# Autodesk Inventor assembly: frame_1_0
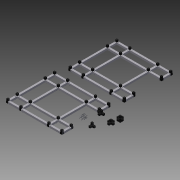
[picture p0: Inventor's stored thumbnail of the model, 180x180]
Saved by Autodesk Inventor 2011 (Build 150239000, 239)
## iProperties
Created: 2013-01-19
Part Number: frame_1_0
Document SubType Name: Assembly
Designer: Christopher
Author: Christopher
## Documents named in this file (30)
- F:\Users\Christopher\Documents\GitHub\2013CAD\2013 robot\forklift\robot_frame\frame_1_0.iam
- F:\Users\Christopher\Documents\GitHub\2013CAD\2013 robot\forklift\robot_frame\tubes_layer1\tube_m_f_in_cross.ipt
- F:\Users\Christopher\Documents\GitHub\2013CAD\2013 robot\forklift\Misc parts\3-way corner.ipt
- F:\Users\Christopher\Documents\GitHub\2013CAD\2013 robot\forklift\Misc parts\4-way corner.ipt
- F:\Users\Christopher\Documents\GitHub\2013CAD\2013 robot\forklift\Misc parts\5-way corner.ipt
- F:\Users\Christopher\Documents\GitHub\2013CAD\2013 robot\forklift\Misc parts\6-way corner.ipt
- F:\Users\Christopher\Documents\GitHub\2013CAD\2013 robot\forklift\Misc parts\1.5_bolt_.25_20.ipt
- F:\Users\Christopher\Documents\GitHub\2013CAD\2013 robot\forklift\robot_frame\tubes_layer1\tube_m_b_in_cross.ipt
- F:\Users\Christopher\Documents\GitHub\2013CAD\2013 robot\forklift\robot_frame\tubes_layer1\tube_m_r_in_mid.ipt
- F:\Users\Christopher\Documents\GitHub\2013CAD\2013 robot\forklift\robot_frame\tubes_layer1\tube_r_b_in.ipt
- F:\Users\Christopher\Documents\GitHub\2013CAD\2013 robot\forklift\robot_frame\tubes_layer1\tube_r_f_in.ipt
- F:\Users\Christopher\Documents\GitHub\2013CAD\2013 robot\forklift\robot_frame\tubes_layer1\tube_m_r_out_center.ipt
- F:\Users\Christopher\Documents\GitHub\2013CAD\2013 robot\forklift\robot_frame\tubes_layer1\tube_b_r_in_wheel.ipt
- F:\Users\Christopher\Documents\GitHub\2013CAD\2013 robot\forklift\robot_frame\tubes_layer1\tube_r_b_out.ipt
- F:\Users\Christopher\Documents\GitHub\2013CAD\2013 robot\forklift\robot_frame\tubes_layer1\tube_b_r_wheel.ipt
- F:\Users\Christopher\Documents\GitHub\2013CAD\2013 robot\forklift\robot_frame\tubes_layer1\tube_f_r_in_wheel.ipt
- F:\Users\Christopher\Documents\GitHub\2013CAD\2013 robot\forklift\robot_frame\tubes_layer1\tube_f_r_out_wheel.ipt
- F:\Users\Christopher\Documents\GitHub\2013CAD\2013 robot\forklift\robot_frame\tubes_layer1\tube_r_f_out.ipt
- F:\Users\Christopher\Documents\GitHub\2013CAD\2013 robot\forklift\robot_frame\tubes_layer1\tube_m_b_out_back.ipt
- F:\Users\Christopher\Documents\GitHub\2013CAD\2013 robot\forklift\robot_frame\tubes_layer1\tube_b_l_in_wheel.ipt
- F:\Users\Christopher\Documents\GitHub\2013CAD\2013 robot\forklift\robot_frame\tubes_layer1\tube_m_l_in.ipt
- F:\Users\Christopher\Documents\GitHub\2013CAD\2013 robot\forklift\robot_frame\tubes_layer1\tube_f_l_in_wheel.ipt
- F:\Users\Christopher\Documents\GitHub\2013CAD\2013 robot\forklift\robot_frame\tubes_layer1\tube_l_f_out.ipt
- F:\Users\Christopher\Documents\GitHub\2013CAD\2013 robot\forklift\robot_frame\tubes_layer1\tube_l_f_in.ipt
- F:\Users\Christopher\Documents\GitHub\2013CAD\2013 robot\forklift\robot_frame\tubes_layer1\tube_l_b_in.ipt
- F:\Users\Christopher\Documents\GitHub\2013CAD\2013 robot\forklift\robot_frame\tubes_layer1\tube_l_b_out.ipt
- F:\Users\Christopher\Documents\GitHub\2013CAD\2013 robot\forklift\robot_frame\tubes_layer1\tube_b_l_out_wheel.ipt
- F:\Users\Christopher\Documents\GitHub\2013CAD\2013 robot\forklift\robot_frame\tubes_layer1\tube_f_l_out_wheel.ipt
- F:\Users\Christopher\Documents\GitHub\2013CAD\2013 robot\forklift\robot_frame\tubes_layer1\tube_m_l_out.ipt
- F:\Users\Christopher\Documents\GitHub\2013CAD\2013 robot\forklift\robot_frame\tubes_layer2\frame_level1_temp.iam
## Components (106 placed, 29 different names)
1. tube_m_f_in_cross:1 — Insert:1, Insert:2, Mate:2, Insert:3, Insert:4, Mate:3
2. 3-way corner:1
3. 4-way corner:1
4. 5-way corner:1
5. 6-way corner:1
6. 5-way corner:2 — Insert:1, Mate:3, Mate:4, Insert:5, Mate:8, Insert:13, Mate:18, Insert:35
7. 1.5_bolt_.25_20:1 — Insert:4
8. 5-way corner:3 — Mate:5, Insert:7, Mate:6, Insert:9, Mate:7, Insert:11, Mate:12, Insert:23
9. 1.5_bolt_.25_20:2 — Insert:2
10. 5-way corner:4 — Mate:2, Insert:3, Mate:30, Insert:58, Mate:31, Insert:62, Mate:34, Insert:70
11. 1.5_bolt_.25_20:3 — Insert:12
12. tube_m_b_in_cross:1 — Mate:6, Insert:9, Insert:10, Mate:25, Insert:49, Insert:51
13. tube_m_r_in_mid:1 — Mate:4, Insert:5, Insert:6, Mate:5, Insert:7, Insert:8
14. 1.5_bolt_.25_20:4 — Insert:6
15. 1.5_bolt_.25_20:5 — Insert:22
16. 1.5_bolt_.25_20:6 — Insert:26
17. 1.5_bolt_.25_20:7 — Insert:28
18. 1.5_bolt_.25_20:8 — Insert:30
19. 1.5_bolt_.25_20:10 — Insert:8
20. 1.5_bolt_.25_20:11 — Insert:10
21. 1.5_bolt_.25_20:12 — Insert:14
22. 1.5_bolt_.25_20:13 — Insert:16
23. 1.5_bolt_.25_20:14 — Insert:18
24. 1.5_bolt_.25_20:15 — Insert:19
25. 1.5_bolt_.25_20:16 — Insert:24
26. tube_r_b_in:1 — Mate:7, Insert:11, Insert:12, Mate:11, Insert:19, Insert:20
27. tube_r_f_in:1 — Mate:8, Insert:13, Insert:14, Mate:9, Insert:15, Insert:16
28. tube_m_r_out_center:1 — Mate:10, Insert:17, Insert:18, Insert:21, Flush:1, Insert:22
29. 4-way corner:2 — Mate:9, Insert:15, Mate:10, Insert:17, Mate:20, Insert:39
30. 4-way corner:3 — Mate:11, Insert:20, Insert:21, Flush:1, Mate:17, Insert:32
31. 3-way corner:2 — Mate:15, Insert:29, Mate:16, Insert:31
32. 4-way corner:4 — Mate:13, Insert:25, Mate:14, Insert:27, Mate:24, Insert:47
33. tube_b_r_in_wheel:1 — Mate:12, Insert:23, Insert:24, Mate:13, Insert:25, Insert:26
34. tube_r_b_out:1 — Mate:14, Insert:27, Insert:28, Mate:15, Insert:29, Insert:30
35. 1.5_bolt_.25_20:17 — Insert:48
36. 1.5_bolt_.25_20:18 — Insert:56
37. 1.5_bolt_.25_20:19 — Insert:42
38. 1.5_bolt_.25_20:20 — Insert:40
39. 1.5_bolt_.25_20:21 — Insert:36
40. 1.5_bolt_.25_20:22 — Insert:51
41. 1.5_bolt_.25_20:23 — Insert:52
42. 1.5_bolt_.25_20:24 — Insert:33
43. 1.5_bolt_.25_20:25 — Insert:45
44. 1.5_bolt_.25_20:26 — Insert:38
45. 1.5_bolt_.25_20:27 — Insert:46
46. 1.5_bolt_.25_20:28 — Insert:34
47. tube_b_r_wheel:1 — Mate:16, Mate:17, Insert:31, Insert:32, Insert:33, Insert:34
48. tube_f_r_in_wheel:1 — Mate:18, Insert:35, Insert:36, Mate:19, Insert:37, Insert:38
49. tube_f_r_out_wheel:1 — Mate:20, Insert:39, Insert:40, Mate:21, Insert:41, Insert:42
50. 3-way corner:3 — Mate:21, Insert:41, Mate:23, Insert:43
51. 3-way corner:4 — Mate:19, Insert:37, Mate:22, Insert:44
52. tube_r_f_out:1 — Mate:22, Mate:23, Insert:43, Insert:44, Insert:45, Insert:46
53. tube_m_b_out_back:1 — Mate:24, Insert:47, Insert:48, Insert:52, Mate:26, Insert:53
54. 5-way corner:5 — Mate:25, Insert:49, Mate:27, Insert:55, Mate:29, Insert:59, Mate:35, Insert:71
55. 4-way corner:5 — Mate:26, Insert:53, Mate:28, Insert:54, Mate:36, Insert:72
56. tube_b_l_in_wheel:1 — Mate:27, Mate:28, Insert:54, Insert:55, Insert:56, Insert:57
57. 1.5_bolt_.25_20:29
58. 1.5_bolt_.25_20:30 — Insert:67
59. 1.5_bolt_.25_20:31 — Insert:69
60. 1.5_bolt_.25_20:32 — Insert:79
61. 1.5_bolt_.25_20:33 — Insert:78
62. 1.5_bolt_.25_20:34 — Insert:63
63. 1.5_bolt_.25_20:35 — Insert:57
64. 1.5_bolt_.25_20:36 — Insert:66
65. 1.5_bolt_.25_20:37 — Insert:61
66. 1.5_bolt_.25_20:38 — Insert:60
67. tube_m_l_in:1 — Mate:29, Mate:30, Insert:58, Insert:59, Insert:60, Insert:61
68. tube_f_l_in_wheel:1 — Mate:31, Insert:62, Insert:63, Mate:32, Insert:64, Insert:67
69. 3-way corner:5 — Mate:32, Insert:64, Flush:2, Insert:65
70. tube_l_f_out:1 — Flush:2, Insert:65, Insert:66, Mate:33, Insert:68, Insert:69
71. 3-way corner:6 — Mate:33, Insert:68, Mate:42, Insert:83
72. tube_l_f_in:1 — Mate:34, Insert:70, Flush:3, Insert:73, Insert:76, Insert:77
73. tube_l_b_in:1 — Mate:35, Insert:71, Flush:4, Insert:74, Insert:78, Insert:93
74. tube_l_b_out:1 — Mate:36, Insert:72, Flush:5, Insert:75, Insert:79, Insert:80
75. 4-way corner:6 — Flush:3, Insert:73, Mate:40, Mate:41, Insert:84, Insert:85
76. 4-way corner:7 — Flush:4, Insert:74, Mate:38, Insert:81, Mate:39, Insert:86, Insert:87
77. 3-way corner:7 — Flush:5, Insert:75, Mate:37, Insert:82, Insert:88
78. 1.5_bolt_.25_20:39 — Insert:76
79. 1.5_bolt_.25_20:40 — Insert:80
80. 1.5_bolt_.25_20:41 — Insert:77
81. 1.5_bolt_.25_20:42 — Insert:93
82. 1.5_bolt_.25_20:43 — Insert:91
83. 1.5_bolt_.25_20:44 — Insert:92
84. 1.5_bolt_.25_20:45 — Insert:90
85. 1.5_bolt_.25_20:46 — Insert:89
86. tube_b_l_out_wheel:1 — Mate:37, Mate:38, Insert:81, Insert:82, Insert:87, Insert:88, Insert:94, Insert:95
87. tube_f_l_out_wheel:1 — Mate:41, Mate:42, Insert:83, Insert:84, Insert:89, Insert:90
88. tube_m_l_out:1 — Mate:39, Mate:40, Insert:85, Insert:86, Insert:91, Insert:92
89. 1.5_bolt_.25_20:47
90. 1.5_bolt_.25_20:48
91. 1.5_bolt_.25_20:49
92. 1.5_bolt_.25_20:50 — Insert:94
93. 1.5_bolt_.25_20:51 — Insert:95
94. 1.5_bolt_.25_20:52
95. 1.5_bolt_.25_20:53
96. 1.5_bolt_.25_20:54
97. 1.5_bolt_.25_20:55
98. 1.5_bolt_.25_20:56
99. 1.5_bolt_.25_20:57
100. 1.5_bolt_.25_20:58
101. 1.5_bolt_.25_20:59
102. 1.5_bolt_.25_20:60
103. 1.5_bolt_.25_20:61
104. 1.5_bolt_.25_20:62
105. 1.5_bolt_.25_20:63
106. frame_level1_temp:1 [sub-assembly]
## Relationships (140: Insert 94, Mate 41, Flush 5)
- Insert:1: tube_m_f_in_cross:1 ↔ 5-way corner:2
- Insert:2: tube_m_f_in_cross:1 ↔ 1.5_bolt_.25_20:2
- Mate:2: tube_m_f_in_cross:1 ↔ 5-way corner:4
- Insert:3: tube_m_f_in_cross:1 ↔ 5-way corner:4
- Insert:4: tube_m_f_in_cross:1 ↔ 1.5_bolt_.25_20:1
- Mate:3: tube_m_f_in_cross:1 ↔ 5-way corner:2
- Mate:4: 5-way corner:2 ↔ tube_m_r_in_mid:1
- Insert:5: 5-way corner:2 ↔ tube_m_r_in_mid:1
- Insert:6: tube_m_r_in_mid:1 ↔ 1.5_bolt_.25_20:4
- Mate:5: 5-way corner:3 ↔ tube_m_r_in_mid:1
- Insert:7: 5-way corner:3 ↔ tube_m_r_in_mid:1
- Insert:8: tube_m_r_in_mid:1 ↔ 1.5_bolt_.25_20:10
- Mate:6: 5-way corner:3 ↔ tube_m_b_in_cross:1
- Insert:9: 5-way corner:3 ↔ tube_m_b_in_cross:1
- Insert:10: tube_m_b_in_cross:1 ↔ 1.5_bolt_.25_20:11
- Mate:7: 5-way corner:3 ↔ tube_r_b_in:1
- Insert:11: 5-way corner:3 ↔ tube_r_b_in:1
- Insert:12: 1.5_bolt_.25_20:3 ↔ tube_r_b_in:1
- Mate:8: 5-way corner:2 ↔ tube_r_f_in:1
- Insert:13: 5-way corner:2 ↔ tube_r_f_in:1
- Insert:14: 1.5_bolt_.25_20:12 ↔ tube_r_f_in:1
- Mate:9: tube_r_f_in:1 ↔ 4-way corner:2
- Insert:15: tube_r_f_in:1 ↔ 4-way corner:2
- Mate:10: tube_m_r_out_center:1 ↔ 4-way corner:2
- Insert:16: 1.5_bolt_.25_20:13 ↔ tube_r_f_in:1
- Insert:17: tube_m_r_out_center:1 ↔ 4-way corner:2
- Insert:18: 1.5_bolt_.25_20:14 ↔ tube_m_r_out_center:1
- Mate:11: tube_r_b_in:1 ↔ 4-way corner:3
- Insert:19: 1.5_bolt_.25_20:15 ↔ tube_r_b_in:1
- Insert:20: tube_r_b_in:1 ↔ 4-way corner:3
- Insert:21: tube_m_r_out_center:1 ↔ 4-way corner:3
- Flush:1: tube_m_r_out_center:1 ↔ 4-way corner:3
- Insert:22: 1.5_bolt_.25_20:5 ↔ tube_m_r_out_center:1
- Mate:12: 5-way corner:3 ↔ tube_b_r_in_wheel:1
- Insert:23: 5-way corner:3 ↔ tube_b_r_in_wheel:1
- Insert:24: 1.5_bolt_.25_20:16 ↔ tube_b_r_in_wheel:1
- Mate:13: 4-way corner:4 ↔ tube_b_r_in_wheel:1
- Insert:25: 4-way corner:4 ↔ tube_b_r_in_wheel:1
- Insert:26: 1.5_bolt_.25_20:6 ↔ tube_b_r_in_wheel:1
- Mate:14: 4-way corner:4 ↔ tube_r_b_out:1
- Insert:27: 4-way corner:4 ↔ tube_r_b_out:1
- Insert:28: 1.5_bolt_.25_20:7 ↔ tube_r_b_out:1
- Mate:15: 3-way corner:2 ↔ tube_r_b_out:1
- Insert:29: 3-way corner:2 ↔ tube_r_b_out:1
- Insert:30: 1.5_bolt_.25_20:8 ↔ tube_r_b_out:1
- Mate:16: 3-way corner:2 ↔ tube_b_r_wheel:1
- Mate:17: 4-way corner:3 ↔ tube_b_r_wheel:1
- Insert:31: 3-way corner:2 ↔ tube_b_r_wheel:1
- Insert:32: 4-way corner:3 ↔ tube_b_r_wheel:1
- Insert:33: 1.5_bolt_.25_20:24 ↔ tube_b_r_wheel:1
- Insert:34: 1.5_bolt_.25_20:28 ↔ tube_b_r_wheel:1
- Mate:18: 5-way corner:2 ↔ tube_f_r_in_wheel:1
- Insert:35: 5-way corner:2 ↔ tube_f_r_in_wheel:1
- Insert:36: 1.5_bolt_.25_20:21 ↔ tube_f_r_in_wheel:1
- Mate:19: tube_f_r_in_wheel:1 ↔ 3-way corner:4
- Insert:37: tube_f_r_in_wheel:1 ↔ 3-way corner:4
- Insert:38: 1.5_bolt_.25_20:26 ↔ tube_f_r_in_wheel:1
- Mate:20: 4-way corner:2 ↔ tube_f_r_out_wheel:1
- Insert:39: 4-way corner:2 ↔ tube_f_r_out_wheel:1
- Insert:40: 1.5_bolt_.25_20:20 ↔ tube_f_r_out_wheel:1
- Mate:21: tube_f_r_out_wheel:1 ↔ 3-way corner:3
- Insert:41: tube_f_r_out_wheel:1 ↔ 3-way corner:3
- Insert:42: 1.5_bolt_.25_20:19 ↔ tube_f_r_out_wheel:1
- Mate:22: 3-way corner:4 ↔ tube_r_f_out:1
- Mate:23: 3-way corner:3 ↔ tube_r_f_out:1
- Insert:43: 3-way corner:3 ↔ tube_r_f_out:1
- Insert:44: 3-way corner:4 ↔ tube_r_f_out:1
- Insert:45: 1.5_bolt_.25_20:25 ↔ tube_r_f_out:1
- Insert:46: 1.5_bolt_.25_20:27 ↔ tube_r_f_out:1
- Mate:24: 4-way corner:4 ↔ tube_m_b_out_back:1
- Insert:47: 4-way corner:4 ↔ tube_m_b_out_back:1
- Insert:48: 1.5_bolt_.25_20:17 ↔ tube_m_b_out_back:1
- Mate:25: tube_m_b_in_cross:1 ↔ 5-way corner:5
- Insert:49: tube_m_b_in_cross:1 ↔ 5-way corner:5
- Insert:51: tube_m_b_in_cross:1 ↔ 1.5_bolt_.25_20:22
- Insert:52: 1.5_bolt_.25_20:23 ↔ tube_m_b_out_back:1
- Mate:26: tube_m_b_out_back:1 ↔ 4-way corner:5
- Insert:53: tube_m_b_out_back:1 ↔ 4-way corner:5
- Mate:27: 5-way corner:5 ↔ tube_b_l_in_wheel:1
- Mate:28: 4-way corner:5 ↔ tube_b_l_in_wheel:1
- Insert:54: 4-way corner:5 ↔ tube_b_l_in_wheel:1
- Insert:55: 5-way corner:5 ↔ tube_b_l_in_wheel:1
- Insert:56: 1.5_bolt_.25_20:18 ↔ tube_b_l_in_wheel:1
- Insert:57: tube_b_l_in_wheel:1 ↔ 1.5_bolt_.25_20:35
- Mate:29: 5-way corner:5 ↔ tube_m_l_in:1
- Mate:30: 5-way corner:4 ↔ tube_m_l_in:1
- Insert:58: 5-way corner:4 ↔ tube_m_l_in:1
- Insert:59: 5-way corner:5 ↔ tube_m_l_in:1
- Insert:60: 1.5_bolt_.25_20:38 ↔ tube_m_l_in:1
- Insert:61: 1.5_bolt_.25_20:37 ↔ tube_m_l_in:1
- Mate:31: 5-way corner:4 ↔ tube_f_l_in_wheel:1
- Insert:62: 5-way corner:4 ↔ tube_f_l_in_wheel:1
- Insert:63: 1.5_bolt_.25_20:34 ↔ tube_f_l_in_wheel:1
- Mate:32: tube_f_l_in_wheel:1 ↔ 3-way corner:5
- Insert:64: tube_f_l_in_wheel:1 ↔ 3-way corner:5
- Flush:2: 3-way corner:5 ↔ tube_l_f_out:1
- Insert:65: 3-way corner:5 ↔ tube_l_f_out:1
- Insert:66: 1.5_bolt_.25_20:36 ↔ tube_l_f_out:1
- Insert:67: 1.5_bolt_.25_20:30 ↔ tube_f_l_in_wheel:1
- Mate:33: tube_l_f_out:1 ↔ 3-way corner:6
- Insert:68: tube_l_f_out:1 ↔ 3-way corner:6
- Insert:69: 1.5_bolt_.25_20:31 ↔ tube_l_f_out:1
- Mate:34: 5-way corner:4 ↔ tube_l_f_in:1
- Mate:35: 5-way corner:5 ↔ tube_l_b_in:1
- Mate:36: 4-way corner:5 ↔ tube_l_b_out:1
- Insert:70: 5-way corner:4 ↔ tube_l_f_in:1
- Insert:71: 5-way corner:5 ↔ tube_l_b_in:1
- Insert:72: 4-way corner:5 ↔ tube_l_b_out:1
- Flush:3: tube_l_f_in:1 ↔ 4-way corner:6
- Flush:4: tube_l_b_in:1 ↔ 4-way corner:7
- Flush:5: tube_l_b_out:1 ↔ 3-way corner:7
- Insert:73: tube_l_f_in:1 ↔ 4-way corner:6
- Insert:74: tube_l_b_in:1 ↔ 4-way corner:7
- Insert:75: tube_l_b_out:1 ↔ 3-way corner:7
- Insert:76: tube_l_f_in:1 ↔ 1.5_bolt_.25_20:39
- Insert:77: tube_l_f_in:1 ↔ 1.5_bolt_.25_20:41
- Insert:78: 1.5_bolt_.25_20:33 ↔ tube_l_b_in:1
- Insert:79: 1.5_bolt_.25_20:32 ↔ tube_l_b_out:1
- Insert:80: tube_l_b_out:1 ↔ 1.5_bolt_.25_20:40
- Mate:37: 3-way corner:7 ↔ tube_b_l_out_wheel:1
- Mate:38: 4-way corner:7 ↔ tube_b_l_out_wheel:1
- Insert:81: 4-way corner:7 ↔ tube_b_l_out_wheel:1
- Insert:82: 3-way corner:7 ↔ tube_b_l_out_wheel:1
- Mate:39: 4-way corner:7 ↔ tube_m_l_out:1
- Mate:40: 4-way corner:6 ↔ tube_m_l_out:1
- Mate:41: 4-way corner:6 ↔ tube_f_l_out_wheel:1
- Mate:42: 3-way corner:6 ↔ tube_f_l_out_wheel:1
- Insert:83: 3-way corner:6 ↔ tube_f_l_out_wheel:1
- Insert:84: 4-way corner:6 ↔ tube_f_l_out_wheel:1
- Insert:85: 4-way corner:6 ↔ tube_m_l_out:1
- Insert:86: 4-way corner:7 ↔ tube_m_l_out:1
- Insert:87: 4-way corner:7 ↔ tube_b_l_out_wheel:1
- Insert:88: 3-way corner:7 ↔ tube_b_l_out_wheel:1
- Insert:89: 1.5_bolt_.25_20:46 ↔ tube_f_l_out_wheel:1
- Insert:90: 1.5_bolt_.25_20:45 ↔ tube_f_l_out_wheel:1
- Insert:91: 1.5_bolt_.25_20:43 ↔ tube_m_l_out:1
- Insert:92: 1.5_bolt_.25_20:44 ↔ tube_m_l_out:1
- Insert:93: tube_l_b_in:1 ↔ 1.5_bolt_.25_20:42
- Insert:94: tube_b_l_out_wheel:1 ↔ 1.5_bolt_.25_20:50
- Insert:95: tube_b_l_out_wheel:1 ↔ 1.5_bolt_.25_20:51
